# Autodesk Inventor assembly: Assembly R2D2
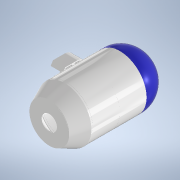
[picture p0: Inventor's stored thumbnail of the model, 180x180]
Saved by Autodesk Inventor 2022.2 (Build 262287010, 287A)
## iProperties
Created: 2022-10-10
Part Number: Assembly R2D2
Document SubType Name: Assembly
Designer: User
Author: User
## Documents named in this file (6)
- C:\Users\User\Videos\R2D2\Partes en 3D\Assembly R2D2.iam
- C:\Users\User\Videos\R2D2\Partes en 3D\Parte media R2D2.ipt
- C:\Users\User\Videos\R2D2\Partes en 3D\Parte baja R2D2.ipt
- C:\Users\User\Videos\R2D2\Partes en 3D\Parte media arriba.ipt
- C:\Users\User\Videos\R2D2\Partes en 3D\Cabeza R2D2.ipt
- C:\Users\User\Videos\R2D2\Partes en 3D\Brazo 3D.ipt
## Components (5 placed, 5 different names)
1. Parte media R2D2:1 — Mate:1, Mate:2
2. Parte baja R2D2:1 — Mate:1
3. Parte media arriba:1 — Mate:2, Mate:3
4. Cabeza R2D2:1 — Mate:3
5. Brazo 3D:1
## Relationships (3: Mate 3)
- Mate:1: Parte media R2D2:1 ↔ Parte baja R2D2:1
- Mate:2: Parte media R2D2:1 ↔ Parte media arriba:1
- Mate:3: Parte media arriba:1 ↔ Cabeza R2D2:1
